# Autodesk Inventor assembly: railFollower
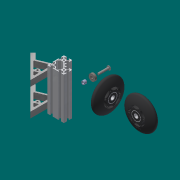
[picture p0: Inventor's stored thumbnail of the model, 180x180]
Saved by Autodesk Inventor 2016 (Build 200138000, 138)
## iProperties
Created: 2016-02-10
Part Number: railFollower
Document SubType Name: Assembly
Designer: Sawaiz
Author: Sawaiz
## Documents named in this file (8)
- C:\Users\Sawaiz\OneDrive\projects\modularRICH\rails\railFollower.iam
- C:\Users\Sawaiz\OneDrive\projects\modularRICH\rails\HFS5-404020-100.ipt
- C:\Users\Sawaiz\OneDrive\projects\modularRICH\rails\MISSION BSX 76MM WHEEL.ipt
- C:\Users\Sawaiz\OneDrive\projects\modularRICH\rails\HBL45TS5hbl45ts5.ipt
- C:\Users\Sawaiz\Desktop\92290A438.ipt
- C:\Users\Sawaiz\OneDrive\projects\modularRICH\testMount\hardware\625BallBearing.ipt
- C:\Users\Sawaiz\OneDrive\projects\modularRICH\testMount\hardware\0.25inSpacer.ipt
- C:\Users\Sawaiz\OneDrive\projects\modularRICH\testMount\hardware\m5x25LowProfile.ipt
## Components (10 placed, 7 different names)
1. HFS5-404020-100:1 — Angle:1, Angle:2, Mate:1, Mate:2, Flush:1, Mate:5, Mate:8, Mate:9
2. MISSION BSX 76MM WHEEL:1 — Angle:1, Mate:3, Mate:4
3. MISSION BSX 76MM WHEEL:2 — Angle:2, Mate:6, Mate:7
4. HBL45TS5hbl45ts5:1 — Mate:1, Mate:2, Flush:1, Flush:2
5. 92290A438:1 — Mate:3, Mate:4, Mate:5
6. 92290A438:2 — Mate:6, Mate:7, Mate:8
7. HBL45TS5hbl45ts5:2 — Mate:9, Flush:2
8. 625BallBearing:1 — Mate:10, Mate:11
9. 0.25inSpacer:1 — Mate:11
10. m5x25LowProfile:1 — Mate:10
## Relationships (15: Mate 11, Angle 2, Flush 2)
- Angle:1 (0 deg): HFS5-404020-100:1 ↔ MISSION BSX 76MM WHEEL:1
- Angle:2 (0 deg): HFS5-404020-100:1 ↔ MISSION BSX 76MM WHEEL:2
- Mate:1: HFS5-404020-100:1 ↔ HBL45TS5hbl45ts5:1
- Mate:2: HFS5-404020-100:1 ↔ HBL45TS5hbl45ts5:1
- Flush:1: HFS5-404020-100:1 ↔ HBL45TS5hbl45ts5:1
- Mate:3: MISSION BSX 76MM WHEEL:1 ↔ 92290A438:1
- Mate:4: MISSION BSX 76MM WHEEL:1 ↔ 92290A438:1
- Mate:5: HFS5-404020-100:1 ↔ 92290A438:1
- Mate:6: MISSION BSX 76MM WHEEL:2 ↔ 92290A438:2
- Mate:7: MISSION BSX 76MM WHEEL:2 ↔ 92290A438:2
- Mate:8: HFS5-404020-100:1 ↔ 92290A438:2
- Mate:9: HFS5-404020-100:1 ↔ HBL45TS5hbl45ts5:2
- Flush:2: HBL45TS5hbl45ts5:1 ↔ HBL45TS5hbl45ts5:2
- Mate:10: 625BallBearing:1 ↔ m5x25LowProfile:1
- Mate:11: 625BallBearing:1 ↔ 0.25inSpacer:1
